# Autodesk Inventor assembly: Tamale - v1p4c
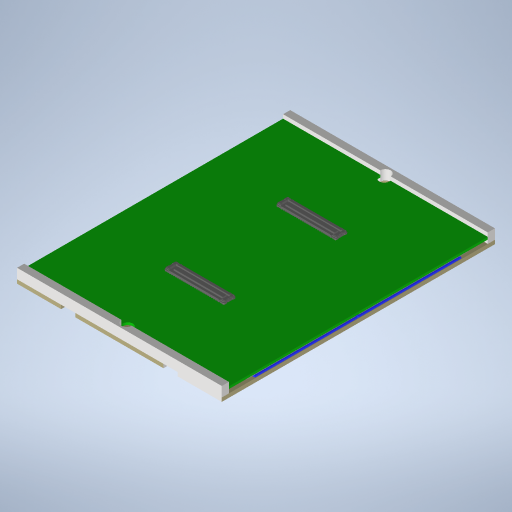
[picture p0: Inventor's stored thumbnail of the model, 512x512]
Saved by Autodesk Inventor 2023 (Build 270158000, 158)
## iProperties
Created: 2022-02-01
Part Number: Tamale - v1p4c
Document SubType Name: Assembly
Designer: Caleb
Author: Caleb
## Documents named in this file (9)
- C:\Users\Caleb\Desktop\nebraska-silicon-lab\Hardware\ETL\modules\tamale v1.4\Tamale - v1p4c.iam
- C:\Users\Caleb\Desktop\nebraska-silicon-lab\Hardware\ETL\modules\tamale v1.4\BBM.iam
- C:\Users\Caleb\Desktop\nebraska-silicon-lab\Hardware\ETL\modules\tamale v1.4\Wirebond.ipt
- C:\Users\Caleb\Desktop\nebraska-silicon-lab\Hardware\ETL\modules\tamale v1.4\Short Wirebond.ipt
- C:\Users\Caleb\Desktop\nebraska-silicon-lab\Hardware\ETL\modules\tamale v1.4\Coverplate Film.ipt
- C:\Users\Caleb\Desktop\nebraska-silicon-lab\Hardware\ETL\modules\tamale v1.4\Sensor Placement Film.ipt
- C:\Users\Caleb\Desktop\nebraska-silicon-lab\Hardware\ETL\modules\tamale v1.4\Baseplate v1.4.ipt
- C:\Users\Caleb\Desktop\nebraska-silicon-lab\Hardware\ETL\modules\tamale v1.4\Mock Module PCB - v1p4c.iam
- C:\Users\Caleb\Desktop\nebraska-silicon-lab\Hardware\ETL\modules\tamale v1.4\block spacer - v1.ipt
## Components (152 placed, 8 different names)
1. BBM:1 [sub-assembly] — Flush:1, Flush:4, Mate:5
2. BBM:2 [sub-assembly] — Flush:2, Flush:4
3. BBM:3 [sub-assembly] — Flush:1, Flush:3, Mate:5, Mate:6, Flush:12
4. BBM:4 [sub-assembly] — Flush:2, Flush:3, Mate:6, Mate:10, Mate:11, Flush:9, Flush:10, Flush:14
5. Mock Module PCB - v1p4c:1 [sub-assembly]
6. Coverplate Film:1 — Mate:10, Flush:12, Flush:14, Mate:12
7. Sensor Placement Film:1 — Mate:11, Flush:9, Flush:10
8. Baseplate v1.4:1 — Mate:12, Mate:13, Flush:16, Flush:17, Mate:14, Flush:18, Flush:19
9. block spacer - v1:1 — Mate:13, Flush:16, Flush:17
10. block spacer - v1:2 — Mate:14, Flush:18, Flush:19
11. Wirebond:143
12. Wirebond:144
13. Wirebond:145
14. Wirebond:146
15. Wirebond:147
16. Wirebond:148
17. Wirebond:149
18. Wirebond:150
19. Wirebond:151
20. Wirebond:152
21. Wirebond:153
22. Wirebond:154
23. Wirebond:155
24. Wirebond:156
25. Wirebond:157
26. Wirebond:158
27. Wirebond:159
28. Wirebond:160
29. Wirebond:161
30. Wirebond:162
31. Wirebond:163
32. Wirebond:164
33. Wirebond:165
34. Wirebond:166
35. Wirebond:167
36. Wirebond:168
37. Wirebond:169
38. Wirebond:170
39. Wirebond:171
40. Wirebond:172
41. Wirebond:173
42. Wirebond:174
43. Wirebond:175
44. Wirebond:176
45. Wirebond:177
46. Wirebond:178
47. Wirebond:179
48. Wirebond:180
49. Wirebond:181
50. Wirebond:182
51. Wirebond:183
52. Wirebond:184
53. Wirebond:185
54. Wirebond:186
55. Wirebond:187
56. Wirebond:188
57. Wirebond:189
58. Wirebond:190
59. Wirebond:191
60. Wirebond:192
61. Wirebond:193
62. Wirebond:194
63. Wirebond:195
64. Wirebond:196
65. Wirebond:197
66. Wirebond:198
67. Wirebond:199
68. Wirebond:200
69. Wirebond:201
70. Wirebond:202
71. Wirebond:203
72. Wirebond:204
73. Wirebond:205
74. Wirebond:206
75. Wirebond:207
76. Wirebond:208
77. Wirebond:209
78. Wirebond:210
79. Wirebond:211
80. Wirebond:212
81. Wirebond:213
82. Short Wirebond:1
83. Short Wirebond:2
84. Short Wirebond:3
85. Short Wirebond:4
86. Short Wirebond:5
87. Short Wirebond:6
88. Short Wirebond:7
89. Short Wirebond:8
90. Short Wirebond:9
91. Short Wirebond:10
92. Short Wirebond:11
93. Short Wirebond:12
94. Short Wirebond:13
95. Short Wirebond:14
96. Short Wirebond:15
97. Short Wirebond:16
98. Short Wirebond:17
99. Short Wirebond:18
100. Short Wirebond:19
101. Short Wirebond:20
102. Short Wirebond:21
103. Short Wirebond:22
104. Short Wirebond:23
105. Short Wirebond:24
106. Short Wirebond:25
107. Short Wirebond:26
108. Short Wirebond:27
109. Short Wirebond:28
110. Short Wirebond:29
111. Short Wirebond:30
112. Short Wirebond:31
113. Short Wirebond:32
114. Short Wirebond:33
115. Short Wirebond:34
116. Short Wirebond:35
117. Short Wirebond:36
118. Short Wirebond:37
119. Short Wirebond:38
120. Short Wirebond:39
121. Short Wirebond:40
122. Short Wirebond:41
123. Short Wirebond:42
124. Short Wirebond:43
125. Short Wirebond:44
126. Short Wirebond:45
127. Short Wirebond:46
128. Short Wirebond:47
129. Short Wirebond:48
130. Short Wirebond:49
131. Short Wirebond:50
132. Short Wirebond:51
133. Short Wirebond:52
134. Short Wirebond:53
135. Short Wirebond:54
136. Short Wirebond:55
137. Short Wirebond:56
138. Short Wirebond:57
139. Short Wirebond:58
140. Short Wirebond:59
141. Short Wirebond:60
142. Short Wirebond:61
143. Short Wirebond:62
144. Short Wirebond:63
145. Short Wirebond:64
146. Short Wirebond:65
147. Short Wirebond:66
148. Short Wirebond:67
149. Short Wirebond:68
150. Short Wirebond:69
151. Short Wirebond:70
152. Short Wirebond:71
## Component patterns: (71 elements, first: Wirebond:143), (71 elements, first: Short Wirebond:1)
## Relationships (25: Flush 14, Mate 11)
- [Mate] (0.08 mm): BBM:3 ↔ Mock Module PCB - v1p4c:1
- [Mate] (0.08 mm): BBM:1 ↔ Mock Module PCB - v1p4c:1
- [Mate] (0.08 mm): BBM:2 ↔ Mock Module PCB - v1p4c:1
- [Mate] (0.08 mm): BBM:4 ↔ Mock Module PCB - v1p4c:1
- Flush:1: BBM:1 ↔ BBM:3
- Flush:2: BBM:2 ↔ BBM:4
- Flush:3: BBM:3 ↔ BBM:4
- Flush:4: BBM:1 ↔ BBM:2
- Mate:5 (0.2 mm): BBM:1 ↔ BBM:3
- Mate:6 (0.2 mm): BBM:3 ↔ BBM:4
- Mate:10: BBM:4 ↔ Coverplate Film:1
- Mate:11: BBM:4 ↔ Sensor Placement Film:1
- Flush:9: BBM:4 ↔ Sensor Placement Film:1
- Flush:10: BBM:4 ↔ Sensor Placement Film:1
- [Flush] (0.25 mm): BBM:1 ↔ Mock Module PCB - v1p4c:1
- Flush:12 (0.5 mm): BBM:3 ↔ Coverplate Film:1
- Flush:14 (0.9 mm): BBM:4 ↔ Coverplate Film:1
- Mate:12: Coverplate Film:1 ↔ Baseplate v1.4:1
- [Flush]: Mock Module PCB - v1p4c:1 ↔ Baseplate v1.4:1
- Mate:13: Baseplate v1.4:1 ↔ block spacer - v1:1
- Flush:16: Baseplate v1.4:1 ↔ block spacer - v1:1
- Flush:17: Baseplate v1.4:1 ↔ block spacer - v1:1
- Mate:14: Baseplate v1.4:1 ↔ block spacer - v1:2
- Flush:18: Baseplate v1.4:1 ↔ block spacer - v1:2
- Flush:19: Baseplate v1.4:1 ↔ block spacer - v1:2
